# Autodesk Inventor assembly: NASA-20-EBOX-EXT-01
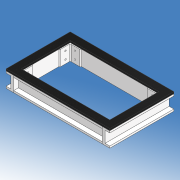
[picture p0: Inventor's stored thumbnail of the model, 180x180]
Saved by Autodesk Inventor 2020 (Build 240168000, 168)
## iProperties
Created: 2019-10-09
Part Number: NASA-20-EBOX-EXT-01
Document SubType Name: Assembly
Designer: mpark
Author: mpark
## Documents named in this file (5)
- C:\Users\mpark\Documents\NASA20\Inventor Files\NASA-20\NASA-20\E-Box\NASA-20-EBOX-EXT-01.iam
- C:\Users\mpark\Documents\NASA20\Inventor Files\NASA-20\NASA-20\E-Box\NASA-20-EBOX-EXTC-01.ipt
- C:\Users\mpark\Documents\NASA20\Inventor Files\NASA-20\NASA-20\E-Box\NASA-20-EBOX-SEXTC-01.ipt
- C:\Users\mpark\Documents\NASA20\Inventor Files\NASA-20\NASA-20\E-Box\Velcro strip.ipt
- C:\Users\mpark\Documents\NASA20\Inventor Files\NASA-20\NASA-20\E-Box\NASA-20-EBOX-EXT-CB-01.ipt
## Components (9 placed, 4 different names)
1. NASA-20-EBOX-EXTC-01:1 — Flush:1, Flush:2, Flush:5, Mate:1, Mate:2, Flush:8, Flush:13, Mate:3, Mate:5
2. NASA-20-EBOX-EXTC-01:2 — Flush:1, Flush:2, Flush:3, Flush:4, Flush:5, Flush:6, Flush:7, Mate:7, Mate:9
3. NASA-20-EBOX-SEXTC-01:1 — Flush:4, Mate:2, Flush:7, Mate:4, Flush:14, Mate:8, Flush:16
4. NASA-20-EBOX-SEXTC-01:2 — Flush:3, Mate:1, Flush:6, Flush:8, Mate:6, Flush:15, Mate:10, Flush:17
5. Velcro strip:1 — Flush:13
6. NASA-20-EBOX-EXT-CB-01:1 — Mate:3, Mate:4, Flush:14
7. NASA-20-EBOX-EXT-CB-01:2 — Mate:7, Mate:8, Flush:16
8. NASA-20-EBOX-EXT-CB-01:3 — Mate:5, Mate:6, Flush:15
9. NASA-20-EBOX-EXT-CB-01:4 — Mate:9, Mate:10, Flush:17
## Relationships (23: Flush 13, Mate 10)
- Flush:1: NASA-20-EBOX-EXTC-01:1 ↔ NASA-20-EBOX-EXTC-01:2
- Flush:2: NASA-20-EBOX-EXTC-01:1 ↔ NASA-20-EBOX-EXTC-01:2
- Flush:3: NASA-20-EBOX-EXTC-01:2 ↔ NASA-20-EBOX-SEXTC-01:2
- Flush:4: NASA-20-EBOX-EXTC-01:2 ↔ NASA-20-EBOX-SEXTC-01:1
- Flush:5: NASA-20-EBOX-EXTC-01:1 ↔ NASA-20-EBOX-EXTC-01:2
- Mate:1: NASA-20-EBOX-EXTC-01:1 ↔ NASA-20-EBOX-SEXTC-01:2
- Mate:2: NASA-20-EBOX-EXTC-01:1 ↔ NASA-20-EBOX-SEXTC-01:1
- Flush:6: NASA-20-EBOX-EXTC-01:2 ↔ NASA-20-EBOX-SEXTC-01:2
- Flush:7: NASA-20-EBOX-EXTC-01:2 ↔ NASA-20-EBOX-SEXTC-01:1
- Flush:8: NASA-20-EBOX-EXTC-01:1 ↔ NASA-20-EBOX-SEXTC-01:2
- Flush:13: NASA-20-EBOX-EXTC-01:1 ↔ Velcro strip:1
- Mate:3: NASA-20-EBOX-EXTC-01:1 ↔ NASA-20-EBOX-EXT-CB-01:1
- Mate:4: NASA-20-EBOX-SEXTC-01:1 ↔ NASA-20-EBOX-EXT-CB-01:1
- Flush:14: NASA-20-EBOX-SEXTC-01:1 ↔ NASA-20-EBOX-EXT-CB-01:1
- Mate:5: NASA-20-EBOX-EXTC-01:1 ↔ NASA-20-EBOX-EXT-CB-01:3
- Mate:6: NASA-20-EBOX-SEXTC-01:2 ↔ NASA-20-EBOX-EXT-CB-01:3
- Flush:15: NASA-20-EBOX-SEXTC-01:2 ↔ NASA-20-EBOX-EXT-CB-01:3
- Mate:7: NASA-20-EBOX-EXTC-01:2 ↔ NASA-20-EBOX-EXT-CB-01:2
- Mate:8: NASA-20-EBOX-SEXTC-01:1 ↔ NASA-20-EBOX-EXT-CB-01:2
- Flush:16: NASA-20-EBOX-SEXTC-01:1 ↔ NASA-20-EBOX-EXT-CB-01:2
- Mate:9: NASA-20-EBOX-EXTC-01:2 ↔ NASA-20-EBOX-EXT-CB-01:4
- Mate:10: NASA-20-EBOX-SEXTC-01:2 ↔ NASA-20-EBOX-EXT-CB-01:4
- Flush:17: NASA-20-EBOX-SEXTC-01:2 ↔ NASA-20-EBOX-EXT-CB-01:4
